# Autodesk Inventor assembly: deployer assy
(part 2 of 2)
- Rigid:381 [WeldJoint]: base plate:1 ↔ 93475A230 M4 Stainless Steel Washer:63
- Rigid:382 [WeldJoint]: base plate:1 ↔ 93475A230 M4 Stainless Steel Washer:60
- Rigid:383 [WeldJoint]: base plate:1 ↔ 93475A230 M4 Stainless Steel Washer:64
- Rigid:384 [WeldJoint]: base plate:1 ↔ 93475A230 M4 Stainless Steel Washer:65
- Rigid:385 [WeldJoint]: base plate:1 ↔ 93475A230 M4 Stainless Steel Washer:66
- Rigid:386 [WeldJoint]: base plate:1 ↔ 93475A230 M4 Stainless Steel Washer:67
- Rigid:387 [WeldJoint]: base plate:1 ↔ 93475A230 M4 Stainless Steel Washer:68
- Rigid:388 [WeldJoint]: 91292A043_18mm 18-8 Stainless Steel Socket Head Screw:48 ↔ 93475A230 M4 Stainless Steel Washer:66
- Rigid:389 [WeldJoint]: 91292A043_18mm 18-8 Stainless Steel Socket Head Screw:47 ↔ 93475A230 M4 Stainless Steel Washer:67
- Rigid:390 [WeldJoint]: 91292A043_18mm 18-8 Stainless Steel Socket Head Screw:46 ↔ 93475A230 M4 Stainless Steel Washer:68
- Rigid:391 [WeldJoint]: 91292A043_18mm 18-8 Stainless Steel Socket Head Screw:45 ↔ 93475A230 M4 Stainless Steel Washer:70
- Rigid:392 [WeldJoint]: 91292A043_18mm 18-8 Stainless Steel Socket Head Screw:44 ↔ 93475A230 M4 Stainless Steel Washer:61
- Rigid:393 [WeldJoint]: 91292A043_18mm 18-8 Stainless Steel Socket Head Screw:43 ↔ 93475A230 M4 Stainless Steel Washer:62
- Mate:23: launch bar:2 ↔ V2.3.1SB:1
- Flush:11: launch bar:2 ↔ V2.3.1SB:1
- Mate:24: mid rack:1 ↔ V2.3.1SB:1
- Mate:25: base plate:1 ↔ PC156-1687-6750-MW-3000-CG-N-IN S:3
- Mate:26: base plate:1 ↔ PC156-1687-6750-MW-3000-CG-N-IN S:3
- Angle:14 (0 deg): base plate:1 ↔ PC156-1687-6750-MW-3000-CG-N-IN S:3
- Mate:27: base plate:1 ↔ PC156-1687-6750-MW-3000-CG-N-IN L:3
- Angle:15 (0 deg): base plate:1 ↔ PC156-1687-6750-MW-3000-CG-N-IN L:3
- Mate:28: base plate:1 ↔ PC156-1687-6750-MW-3000-CG-N-IN L:3
- Mate:29: launch bar:1 ↔ V2.3.1SB:100
- Flush:12: launch bar:1 ↔ V2.3.1SB:100
- Mate:30: front rack 2:1 ↔ V2.3.1SB:100
- Rigid:395 [WeldJoint]: stilt connector F:1 ↔ M83513_03-F03N:1
